# Autodesk Inventor assembly: A_Flightcontroller_PCB
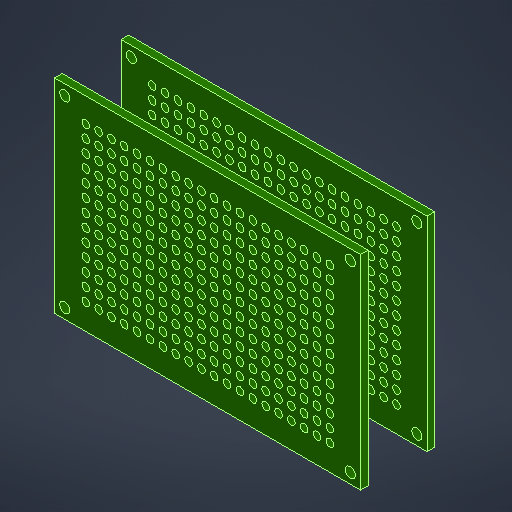
[picture p0: Inventor's stored thumbnail of the model, 512x512]
Saved by Autodesk Inventor 2026 (Build 300175000, 175)
## iProperties
Created: 2025-09-06
Part Number: A_Flightcontroller_PCB
Document SubType Name: Assembly
Designer: FAL
Author: FAL
## Documents named in this file (3)
- C:\Users\FAL\Projekte\Git\AEROLAB\01_AIRCRAFTS\AIR-BERT\CAD\A_Flightcontroller_PCB.iam
- C:\Users\FAL\Projekte\Git\AEROLAB\01_AIRCRAFTS\AIR-BERT\CAD\P_PCB_40x60.ipt
- C:\Users\FAL\Projekte\Git\AEROLAB\01_AIRCRAFTS\AIR-BERT\CAD\extern\XIAO-ESP32S3 v2.iam
## Components (3 placed, 2 different names)
1. P_PCB_40x60:1 — Fluchtend:1, Fluchtend:2, Passend:1, Fluchtend:5, Fluchtend:6, Fluchtend:7
2. XIAO-ESP32S3 v2:1 [sub-assembly] — Passend:1
3. P_PCB_40x60:2 — Fluchtend:3, Fluchtend:4
## Relationships (8: Flush 7, Mate 1)
- Fluchtend:1 [Flush]: P_PCB_40x60:1
- Fluchtend:2 [Flush]: P_PCB_40x60:1
- Passend:1 [Mate]: P_PCB_40x60:1 ↔ XIAO-ESP32S3 v2:1
- Fluchtend:3 [Flush]: P_PCB_40x60:2
- Fluchtend:4 [Flush]: P_PCB_40x60:2
- Fluchtend:5 [Flush]: P_PCB_40x60:1
- Fluchtend:6 [Flush]: P_PCB_40x60:1
- Fluchtend:7 [Flush]: P_PCB_40x60:1
